# Autodesk Inventor assembly: HS 36T Gear, Square_MIR3
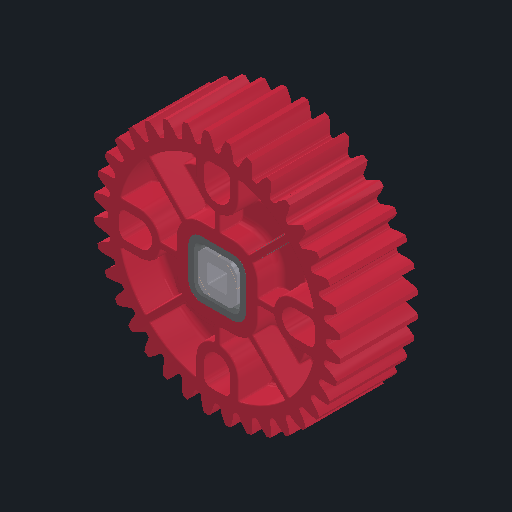
[picture p0: Inventor's stored thumbnail of the model, 512x512]
Saved by Autodesk Inventor 2023 (Build 270158000, 158)
## iProperties
Created: 2022-08-02
Part Number: HS 36T Gear, Square_MIR3
Document SubType Name: Assembly
Designer: Windows Macbook
Author: ylu12
## Documents named in this file (3)
- C:\Users\Windows Macbook\Desktop\VRC-SPIN-UP\Inventor\Motion\Gears\HS Gear\HS 36T Gear, Square_MIR3.iam
- C:\Users\Windows Macbook\Desktop\VRC-SPIN-UP\Inventor\Motion\HS Shaft Adapter Square_MIR3.ipt
- C:\Users\Windows Macbook\Desktop\VRC-SPIN-UP\Inventor\Motion\Gears\Reference Files\HS 36T Gear, No Insert_MIR3.ipt
## Components (2 placed, 2 different names)
1. HS Shaft Adapter Square_MIR3:1 — Flush:2, Mate:4, Mate:3
2. HS 36T Gear, No Insert_MIR3:1 — Mate:10, Mate:9, Flush:5
## Relationships (6: Mate 4, Flush 2)
- Flush:2 (-6.35 mm): HS Shaft Adapter Square_MIR3:1
- Mate:4: HS Shaft Adapter Square_MIR3:1
- Mate:3: HS Shaft Adapter Square_MIR3:1
- Mate:10: HS 36T Gear, No Insert_MIR3:1
- Mate:9: HS 36T Gear, No Insert_MIR3:1
- Flush:5: HS 36T Gear, No Insert_MIR3:1
